# Autodesk Inventor assembly: 316-02
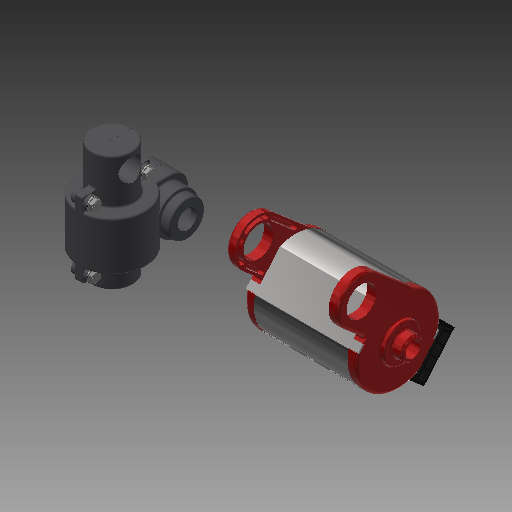
[picture p0: Inventor's stored thumbnail of the model, 512x512]
Saved by Autodesk Inventor 2019 (Build 230136000, 136)
## iProperties
Company: Autodesk Inc.
Created: 2008-01-21
Part Number: 316-02
Document SubType Name: Assembly
Designer: Autodesk Inc.
Mass: 126.589 g
Surface Area: 610.96 cm^2
Volume: 70.4052 cm^3
Density: 1.798 g/cm^3
Author: Inventor
## Documents named in this file (5)
- C:\TEMP\Car Seat\Workspace\Front Drive Assembly.iam
- C:\TEMP\Car Seat\Workspace\Motor.iam
- C:\TEMP\Car Seat\Workspace\Gear Housing Case L.ipt
- C:\TEMP\Car Seat\Workspace\Gear Housing Case R.ipt
- C:\TEMP\Car Seat\Workspace\AS 1417 - Metric M3 x 6.ipt
## Components (7 placed, 4 different names)
1. Gear Housing Case L:1 — Mate:1, Mate:12, Mate:3, Insert:1, Insert:2, Insert:3, Insert:4, Mate:11, Mate:10, Mate:9
2. AS 1427 - Metric M3 x 6:5 — Insert:1
3. AS 1427 - Metric M3 x 6:6 — Insert:2
4. AS 1427 - Metric M3 x 6:7 — Insert:3
5. AS 1427 - Metric M3 x 6:8 — Insert:4
6. Gear Housing Case R:1 — Mate:1, Mate:12, Mate:3
7. Motor:1 [sub-assembly] — Mate:11, Mate:10, Mate:9
## Relationships (10: Mate 6, Insert 4)
- Mate:1: Gear Housing Case L:1 ↔ Gear Housing Case R:1
- Mate:12: Gear Housing Case L:1 ↔ Gear Housing Case R:1
- Mate:3: Gear Housing Case L:1 ↔ Gear Housing Case R:1
- Insert:1: Gear Housing Case L:1 ↔ AS 1427 - Metric M3 x 6:5
- Insert:2: Gear Housing Case L:1 ↔ AS 1427 - Metric M3 x 6:6
- Insert:3: Gear Housing Case L:1 ↔ AS 1427 - Metric M3 x 6:7
- Insert:4: Gear Housing Case L:1 ↔ AS 1427 - Metric M3 x 6:8
- Mate:11: Gear Housing Case L:1 ↔ Motor:1
- Mate:10: Gear Housing Case L:1 ↔ Motor:1
- Mate:9 (45.5 mm): Gear Housing Case L:1 ↔ Motor:1
